# Autodesk Inventor assembly: Second Base Extension (Foraging Arm)
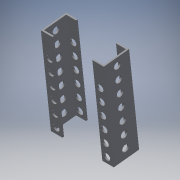
[picture p0: Inventor's stored thumbnail of the model, 180x180]
Saved by Autodesk Inventor 2018 (Build 220112000, 112)
## iProperties
Created: 2017-07-14
Part Number: Second Base Extension (Foraging Arm)
Document SubType Name: Assembly
Designer: James
Author: James
## Documents named in this file (2)
- C:\Users\James\Desktop\EE REU\Hardware\Vex Arm\Vex Arm Draft 2\Second Base Extension (Foraging Arm).iam
- C:\Users\James\Desktop\EE REU\Hardware\Vex Arm\Vex Parts\Base C Channel.ipt
## Components (2 placed, 1 different names)
1. Base C Channel:1
2. Base C Channel:2
## Relationships (3: Flush 2, Mate 1)
- [Mate] (60 mm): Base C Channel:1 ↔ Base C Channel:2
- [Flush]: Base C Channel:1 ↔ Base C Channel:2
- [Flush]: Base C Channel:1 ↔ Base C Channel:2
